# Autodesk Inventor assembly: A2017_T2_04
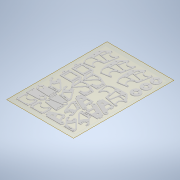
[picture p0: Inventor's stored thumbnail of the model, 180x180]
Saved by Autodesk Inventor 2020 (Build 240168000, 168)
## iProperties
Created: 2021-08-27
Part Number: A2017_T2_04
Document SubType Name: Assembly
Designer: Masato
Author: Masato
## Documents named in this file (10)
- C:\Users\L20C1118 森　圭汰\Documents\20220327_open\SUSTAINA-OP\Cam\A2017_T2_04.iam
- C:\Users\L20C1118 森　圭汰\Documents\20220327_open\SUSTAINA-OP\Cam\DisposableBoard.ipt
- C:\Users\L20C1118 森　圭汰\Documents\20220327_open\SUSTAINA-OP\LowerBody\Foot\Foot_front_frame.ipt
- C:\Users\L20C1118 森　圭汰\Documents\20220327_open\SUSTAINA-OP\LowerBody\Foot\Foot_back_frame.ipt
- C:\Users\L20C1118 森　圭汰\Documents\20220327_open\SUSTAINA-OP\LowerBody\Ankle\Ankle_back_frame.ipt
- C:\Users\L20C1118 森　圭汰\Documents\20220327_open\SUSTAINA-OP\UpperBody\Trunk\CrossRollerBearing\Inner_flange.ipt
- C:\Users\L20C1118 森　圭汰\Documents\20220327_open\SUSTAINA-OP\LowerBody\Ankle\Ankle_side_frame.ipt
- C:\Users\L20C1118 森　圭汰\Documents\20220327_open\SUSTAINA-OP\LowerBody\Knee\Knee_side_frame.ipt
- C:\Users\L20C1118 森　圭汰\Documents\20220327_open\SUSTAINA-OP\LowerBody\Leg_joint\Leg_joint_pitch_frame.ipt
- C:\Users\L20C1118 森　圭汰\Documents\20220327_open\SUSTAINA-OP\UpperBody\Arm\Shoulder_side_frame.ipt
## Components (25 placed, 9 different names)
1. DisposableBoard:1 — メイト:2, メイト:1, フラッシュ:1, フラッシュ:2, メイト:4, メイト:5, メイト:6, メイト:7, メイト:8, メイト:9, フラッシュ:3, フラッシュ:4, フラッシュ:5, 正接:1, 角度:1, メイト:20, メイト:22, メイト:23, フラッシュ:7, メイト:27, メイト:28, 正接:9, フラッシュ:8, メイト:32, メイト:33, 正接:12, メイト:36, フラッシュ:10, メイト:38, メイト:39, 正接:17, フラッシュ:11, 角度:2, 正接:21, 正接:22, メイト:47, メイト:50, フラッシュ:12, 角度:3
2. Foot_back_frame:1 — メイト:7, メイト:10, フラッシュ:5, メイト:11
3. Foot_back_frame:2 — メイト:8, 正接:1, メイト:11, メイト:14, メイト:29
4. Foot_front_frame:2 — メイト:6, メイト:12, メイト:13, 角度:1, 正接:4
5. Foot_front_frame:1 — メイト:5, メイト:13, メイト:14, 正接:4, メイト:30
6. Leg_joint_pitch_frame:1 — メイト:22, フラッシュ:8, メイト:31, 正接:14, メイト:40
7. Leg_joint_pitch_frame:2 — メイト:23, 正接:14, メイト:45, メイト:49
8. Shoulder_side_frame:1 — メイト:27, メイト:29, 正接:9, 正接:11
9. Shoulder_side_frame:2 — メイト:28, メイト:30, 正接:11
10. Shoulder_side_frame:3 — メイト:32, 正接:19, フラッシュ:11, メイト:42
11. Shoulder_side_frame:4 — メイト:31, メイト:33, 正接:12, メイト:42
12. Leg_joint_pitch_frame:3 — メイト:36, フラッシュ:10, メイト:41, 正接:19, メイト:48
13. Leg_joint_pitch_frame:4 — メイト:38, メイト:40, 正接:17, メイト:43
14. Knee_side_frame:4 — メイト:39, 角度:2, 正接:20, 正接:23, メイト:43
15. Shoulder_side_frame:5 — メイト:47, メイト:48, メイト:49
16. Ankle_back_frame:1 — メイト:4, フラッシュ:3, フラッシュ:4, メイト:10
17. Ankle_back_frame:2 — メイト:12, メイト:41
18. Ankle_side_frame:1 — メイト:20, フラッシュ:7, メイト:45
19. Ankle_side_frame:2 — 正接:20, 正接:23, 正接:24
20. Knee_side_frame:1 — メイト:50, フラッシュ:12, 正接:24
21. Knee_side_frame:5
22. Knee_side_frame:6
23. Inner_flange:1 — メイト:9, 正接:21, 正接:22, 角度:3
24. Inner_flange:2
25. Inner_flange:3
## Component patterns: (2 elements, first: Ankle_back_frame:1), (2 elements, first: Ankle_side_frame:1), (3 elements, first: Knee_side_frame:1), (3 elements, first: Inner_flange:1)
## Relationships (61: Mate 35, Tangent 13, Flush 10, Angle 3)
- メイト:2 [Mate]: DisposableBoard:1
- メイト:1 [Mate]: DisposableBoard:1
- フラッシュ:1 [Flush]: DisposableBoard:1
- フラッシュ:2 [Flush]: DisposableBoard:1
- メイト:4 [Mate]: DisposableBoard:1 ↔ Ankle_back_frame:1
- メイト:5 [Mate]: DisposableBoard:1 ↔ Foot_front_frame:1
- メイト:6 [Mate]: DisposableBoard:1 ↔ Foot_front_frame:2
- メイト:7 [Mate]: DisposableBoard:1 ↔ Foot_back_frame:1
- メイト:8 [Mate]: DisposableBoard:1 ↔ Foot_back_frame:2
- メイト:9 [Mate]: DisposableBoard:1 ↔ Inner_flange:1
- フラッシュ:3 [Flush] (2 mm): DisposableBoard:1 ↔ Ankle_back_frame:1
- フラッシュ:4 [Flush] (2 mm): DisposableBoard:1 ↔ Ankle_back_frame:1
- メイト:10 [Mate] (2.5 mm): Foot_back_frame:1 ↔ Ankle_back_frame:1
- フラッシュ:5 [Flush] (2 mm): DisposableBoard:1 ↔ Foot_back_frame:1
- 正接:1 [Tangent] (2 mm): DisposableBoard:1 ↔ Foot_back_frame:2
- メイト:11 [Mate] (2.5 mm): Foot_back_frame:1 ↔ Foot_back_frame:2
- メイト:12 [Mate] (2.5 mm): Foot_front_frame:2 ↔ Ankle_back_frame:2
- メイト:13 [Mate] (2.5 mm): Foot_front_frame:2 ↔ Foot_front_frame:1
- 角度:1 [Angle] (180 deg): DisposableBoard:1 ↔ Foot_front_frame:2
- メイト:14 [Mate] (2.5 mm): Foot_back_frame:2 ↔ Foot_front_frame:1
- 正接:4 [Tangent]: Foot_front_frame:2 ↔ Foot_front_frame:1
- メイト:20 [Mate]: DisposableBoard:1 ↔ Ankle_side_frame:1
- メイト:22 [Mate]: DisposableBoard:1 ↔ Leg_joint_pitch_frame:1
- メイト:23 [Mate]: DisposableBoard:1 ↔ Leg_joint_pitch_frame:2
- フラッシュ:7 [Flush] (2 mm): DisposableBoard:1 ↔ Ankle_side_frame:1
- メイト:27 [Mate]: DisposableBoard:1 ↔ Shoulder_side_frame:1
- メイト:28 [Mate]: DisposableBoard:1 ↔ Shoulder_side_frame:2
- メイト:29 [Mate] (2.5 mm): Foot_back_frame:2 ↔ Shoulder_side_frame:1
- 正接:9 [Tangent] (2 mm): DisposableBoard:1 ↔ Shoulder_side_frame:1
- メイト:30 [Mate] (2.5 mm): Foot_front_frame:1 ↔ Shoulder_side_frame:2
- 正接:11 [Tangent] (2.5 mm): Shoulder_side_frame:1 ↔ Shoulder_side_frame:2
- フラッシュ:8 [Flush] (2 mm): DisposableBoard:1 ↔ Leg_joint_pitch_frame:1
- メイト:31 [Mate] (2.5 mm): Leg_joint_pitch_frame:1 ↔ Shoulder_side_frame:4
- メイト:32 [Mate]: DisposableBoard:1 ↔ Shoulder_side_frame:3
- メイト:33 [Mate]: DisposableBoard:1 ↔ Shoulder_side_frame:4
- 正接:12 [Tangent] (2 mm): DisposableBoard:1 ↔ Shoulder_side_frame:4
- 正接:14 [Tangent] (2.5 mm): Leg_joint_pitch_frame:1 ↔ Leg_joint_pitch_frame:2
- メイト:36 [Mate]: DisposableBoard:1 ↔ Leg_joint_pitch_frame:3
- フラッシュ:10 [Flush] (2 mm): DisposableBoard:1 ↔ Leg_joint_pitch_frame:3
- メイト:38 [Mate]: DisposableBoard:1 ↔ Leg_joint_pitch_frame:4
- メイト:39 [Mate]: DisposableBoard:1 ↔ Knee_side_frame:4
- メイト:40 [Mate] (2.5 mm): Leg_joint_pitch_frame:1 ↔ Leg_joint_pitch_frame:4
- 正接:17 [Tangent] (2 mm): DisposableBoard:1 ↔ Leg_joint_pitch_frame:4
- メイト:41 [Mate] (2.5 mm): Leg_joint_pitch_frame:3 ↔ Ankle_back_frame:2
- 正接:19 [Tangent] (2.5 mm): Shoulder_side_frame:3 ↔ Leg_joint_pitch_frame:3
- フラッシュ:11 [Flush] (2 mm): DisposableBoard:1 ↔ Shoulder_side_frame:3
- メイト:42 [Mate] (2.5 mm): Shoulder_side_frame:3 ↔ Shoulder_side_frame:4
- 角度:2 [Angle] (0 deg): DisposableBoard:1 ↔ Knee_side_frame:4
- 正接:20 [Tangent] (2.5 mm): Knee_side_frame:4 ↔ Ankle_side_frame:2
- 正接:21 [Tangent] (2 mm): DisposableBoard:1 ↔ Inner_flange:1
- 正接:22 [Tangent] (2 mm): DisposableBoard:1 ↔ Inner_flange:1
- 正接:23 [Tangent] (2.5 mm): Knee_side_frame:4 ↔ Ankle_side_frame:2
- メイト:43 [Mate] (2.5 mm): Leg_joint_pitch_frame:4 ↔ Knee_side_frame:4
- メイト:45 [Mate] (2.5 mm): Leg_joint_pitch_frame:2 ↔ Ankle_side_frame:1
- メイト:47 [Mate]: DisposableBoard:1 ↔ Shoulder_side_frame:5
- メイト:48 [Mate] (2.5 mm): Leg_joint_pitch_frame:3 ↔ Shoulder_side_frame:5
- メイト:49 [Mate] (2.5 mm): Leg_joint_pitch_frame:2 ↔ Shoulder_side_frame:5
- メイト:50 [Mate]: DisposableBoard:1 ↔ Knee_side_frame:1
- フラッシュ:12 [Flush] (2 mm): DisposableBoard:1 ↔ Knee_side_frame:1
- 正接:24 [Tangent] (2.5 mm): Ankle_side_frame:2 ↔ Knee_side_frame:1
- 角度:3 [Angle] (0 deg): DisposableBoard:1 ↔ Inner_flange:1
